# Autodesk Inventor assembly: Camera
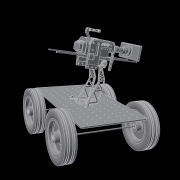
[picture p0: Inventor's stored thumbnail of the model, 180x180]
Saved by Autodesk Inventor 2020.4 (Build 244396010, 396A)
## iProperties
Created: 2022-09-19
Part Number: Camera
Document SubType Name: Assembly
Designer: Val
Author: Val
## Documents named in this file (11)
- C:\Users\Val\Desktop\tau\quote\Camera.iam
- C:\Users\Val\Desktop\tau\quote\Body.ipt
- C:\Users\Val\Desktop\tau\quote\BodyMirror.ipt
- C:\Users\Val\Desktop\tau\quote\S1.ipt
- C:\Users\Val\Desktop\tau\quote\S2.ipt
- C:\Users\Val\Desktop\tau\quote\CameraBody.ipt
- C:\Users\Val\Downloads\2481T51_Rubber Solid-Tread Flat-Free Wheel on Aluminum Core.ipt
- C:\Users\Val\Desktop\tau\external\TopHandle.ipt
- C:\Users\Val\Desktop\tau\MuzzleTube.ipt
- C:\Users\Val\Desktop\drummingrobot\src\parts\TorsoMount.ipt
- C:\Users\Val\Desktop\tau\quote\Part4.ipt
## Components (16 placed, 13 different names)
1. Body:1 — Flush:2, Flush:3, Mate:11, Mate:32, Flush:11
2. BodyMirror:1 — Flush:2, Flush:3, Mate:12, Mate:33
3. S1:1 — Mate:13, Flush:4, Mate:15, Angle:3
4. S2:1 — Mate:14, Flush:4, Mate:15, Mate:34
5. CameraBody:1 — Mate:11, Mate:12, Mate:13, Mate:14, Mate:17, Angle:1, Angle:3, Flush:11, Mate:35
6. 2481T51_Rubber Solid-Tread Flat-Free Wheel on Aluminum Core:1 — Mate:29, Flush:6, Flush:12
7. 2481T51_Rubber Solid-Tread Flat-Free Wheel on Aluminum Core:2 — Mate:28, Flush:7
8. 2481T51_Rubber Solid-Tread Flat-Free Wheel on Aluminum Core:3 — Mate:30, Flush:9, Flush:12
9. 2481T51_Rubber Solid-Tread Flat-Free Wheel on Aluminum Core:4 — Mate:31, Flush:8
10. TopHandle:1 — Mate:17, Angle:1, Mate:35
11. MT1 — Mate:28, Mate:29, Flush:6, Flush:7, Angle:4
12. MT2 — Mate:30, Mate:31, Flush:8, Flush:9
13. MT3 — Mate:32, Flush:10
14. MT4 — Mate:33, Flush:10
15. TMount — Mate:34
16. Part4:1 — Angle:4
## Relationships (27: Mate 14, Flush 10, Angle 3)
- Flush:2: Body:1 ↔ BodyMirror:1
- Flush:3: Body:1 ↔ BodyMirror:1
- Mate:11: Body:1 ↔ CameraBody:1
- Mate:12: BodyMirror:1 ↔ CameraBody:1
- Mate:13: S1:1 ↔ CameraBody:1
- Mate:14: S2:1 ↔ CameraBody:1
- Flush:4: S1:1 ↔ S2:1
- Mate:15: S1:1 ↔ S2:1
- Mate:17: CameraBody:1 ↔ TopHandle:1
- Angle:1 (0 deg): CameraBody:1 ↔ TopHandle:1
- Mate:28: 2481T51_Rubber Solid-Tread Flat-Free Wheel on Aluminum Core:2 ↔ MT1
- Mate:29: 2481T51_Rubber Solid-Tread Flat-Free Wheel on Aluminum Core:1 ↔ MT1
- Flush:6: 2481T51_Rubber Solid-Tread Flat-Free Wheel on Aluminum Core:1 ↔ MT1
- Flush:7: 2481T51_Rubber Solid-Tread Flat-Free Wheel on Aluminum Core:2 ↔ MT1
- Mate:30: 2481T51_Rubber Solid-Tread Flat-Free Wheel on Aluminum Core:3 ↔ MT2
- Mate:31: 2481T51_Rubber Solid-Tread Flat-Free Wheel on Aluminum Core:4 ↔ MT2
- Flush:8: 2481T51_Rubber Solid-Tread Flat-Free Wheel on Aluminum Core:4 ↔ MT2
- Flush:9: 2481T51_Rubber Solid-Tread Flat-Free Wheel on Aluminum Core:3 ↔ MT2
- Mate:32: Body:1 ↔ MT3
- Mate:33: BodyMirror:1 ↔ MT4
- Mate:34: S2:1 ↔ TMount
- Flush:10: MT3 ↔ MT4
- Angle:3 (0 deg): S1:1 ↔ CameraBody:1
- Flush:11: Body:1 ↔ CameraBody:1
- Flush:12: 2481T51_Rubber Solid-Tread Flat-Free Wheel on Aluminum Core:1 ↔ 2481T51_Rubber Solid-Tread Flat-Free Wheel on Aluminum Core:3
- Mate:35: CameraBody:1 ↔ TopHandle:1
- Angle:4 (0 deg): MT1 ↔ Part4:1
